# Autodesk Inventor assembly: Extruder 2.3
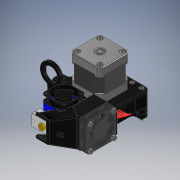
[picture p0: Inventor's stored thumbnail of the model, 180x180]
Saved by Autodesk Inventor 2020.2 (Build 242310000, 310)
## iProperties
Created: 2020-03-20
Part Number: Extruder 2.3
Document SubType Name: Assembly
Designer: rah75
Author: rah75
## Documents named in this file (29)
- C:\Users\rah75\Documents\GitHub\LETU-Maker\CAD\Autodesk Inventor\Modules_6001-9999\Extruder\Assemblies\Extruder_LM6012.iam
- C:\Users\rah75\Documents\GitHub\LETU-Maker\CAD\Autodesk Inventor\Modules_6001-9999\Extruder\Printed_Parts\Extruder_Lower_Block_LM6008.ipt
- C:\Users\rah75\Documents\GitHub\LETU-Maker\CAD\Autodesk Inventor\Modules_6001-9999\Extruder\Printed_Parts\Extruder_Motor_Plate_LM6009.ipt
- C:\Users\rah75\Documents\GitHub\LETU-Maker\CAD\Autodesk Inventor\Modules_6001-9999\Extruder\Printed_Parts\Extruder_Upper_Block_LM6011.ipt
- C:\Users\rah75\Documents\GitHub\LETU-Maker\CAD\Autodesk Inventor\Modules_6001-9999\Extruder\Printed_Parts\Extruder_Mount_Plate_LM6010.ipt
- C:\Users\rah75\Documents\GitHub\LETU-Maker\CAD\Autodesk Inventor\Stock_Components_1001-2999\Misc\Hot_End_Plate_LM1038.ipt
- C:\Users\rah75\Documents\GitHub\LETU-Maker\CAD\Autodesk Inventor\Stock_Components_1001-2999\Motors\NEMA_17_LM1028.ipt
- C:\Users\rah75\Documents\GitHub\LETU-Maker\CAD\Autodesk Inventor\Modules_6001-9999\Extruder\Printed_Parts\Extruder_Gear_0.8m57t_Internal_LM6004.ipt
- C:\Users\rah75\Documents\GitHub\LETU-Maker\CAD\Autodesk Inventor\Stock_Components_1001-2999\Power_Transmission\Bearings\625-ZZ_5x16mm_LM1030.ipt
- C:\Users\rah75\Documents\GitHub\LETU-Maker\CAD\Autodesk Inventor\Stock_Components_1001-2999\Power_Transmission\extruder_knob_11mm_LM1033.ipt
- C:\Users\rah75\Documents\GitHub\LETU-Maker\CAD\Autodesk Inventor\Modules_6001-9999\Extruder\Fabricated_Parts\Extruder_Fillament_Guide_LM6002.ipt
- C:\Users\rah75\Documents\GitHub\LETU-Maker\CAD\Autodesk Inventor\Stock_Components_1001-2999\Electrical\e3d-v6-hotend-3\e3d v6.iam
- C:\Users\rah75\Documents\GitHub\LETU-Maker\CAD\Autodesk Inventor\Modules_6001-9999\Extruder\Printed_Parts\Extruder_Pinion_0.8m12t_LM6005.ipt
- C:\Users\rah75\Documents\GitHub\LETU-Maker\CAD\Autodesk Inventor\Modules_6001-9999\Extruder\Fabricated_Parts\Extruder_Drive_Shaft_LM6001.ipt
- C:\Users\rah75\Documents\GitHub\LETU-Maker\CAD\Autodesk Inventor\Modules_6001-9999\Extruder\Fabricated_Parts\Extruder_Idler_Shaft_LM6003.ipt
- C:\Users\rah75\Documents\GitHub\LETU-Maker\CAD\Autodesk Inventor\Stock_Components_1001-2999\Fasteners\Screws\SHCS_m3x20_LM1014.ipt
- C:\Users\rah75\Documents\GitHub\LETU-Maker\CAD\Autodesk Inventor\Stock_Components_1001-2999\Fasteners\Screws\SHCS_m3x35_LM1011.ipt
- C:\Users\rah75\Documents\GitHub\LETU-Maker\CAD\Autodesk Inventor\Modules_6001-9999\Extruder\Printed_Parts\Extruder_Inductive_Sensor_Mount_LM6007.ipt
- C:\Users\rah75\Documents\GitHub\LETU-Maker\CAD\Autodesk Inventor\Stock_Components_1001-2999\Electrical\fan_40x40mm_LM1027.ipt
- C:\Users\rah75\Documents\GitHub\LETU-Maker\CAD\Autodesk Inventor\Stock_Components_1001-2999\Fasteners\Nuts\heat_insert_m3_LM1017.ipt
- C:\Users\rah75\Documents\GitHub\LETU-Maker\CAD\Autodesk Inventor\Stock_Components_1001-2999\Fasteners\Screws\SHCS_m3x8_LM1008.ipt
- C:\Users\rah75\Documents\GitHub\LETU-Maker\CAD\Autodesk Inventor\Stock_Components_1001-2999\Fasteners\Screws\SHCS_m3x10_LM1015.ipt
- C:\Users\rah75\Documents\GitHub\LETU-Maker\CAD\Autodesk Inventor\Stock_Components_1001-2999\Fasteners\Screws\SHCS_m3x30_LM1012.ipt
- C:\Users\rah75\Documents\GitHub\LETU-Maker\CAD\Autodesk Inventor\Stock_Components_1001-2999\Fasteners\Screws\SHCS_m3x12_LM1037.ipt
- C:\Users\rah75\Documents\GitHub\LETU-Maker\CAD\Autodesk Inventor\Stock_Components_1001-2999\Fasteners\Nuts\hex_nut_m3_LM1019.ipt
- C:\Users\rah75\Documents\GitHub\LETU-Maker\CAD\Autodesk Inventor\Stock_Components_1001-2999\Fasteners\Screws\Set Screws\set_screw_m3x6_LM1016.ipt
- C:\Users\rah75\Documents\GitHub\LETU-Maker\CAD\Autodesk Inventor\Stock_Components_1001-2999\Fasteners\Screws\SHCS_m3x5_LM1007.ipt
- C:\Users\rah75\Documents\GitHub\LETU-Maker\CAD\Autodesk Inventor\Modules_6001-9999\Extruder\Printed_Parts\Extruder_Fan_Duct_LM6006.ipt
- C:\Users\rah75\Documents\GitHub\LETU-Maker\CAD\Autodesk Inventor\Modules_6001-9999\Extruder\Printed_Parts\Extruder_Hot_End_Spacer_LM6014.ipt
## Components (50 placed, 28 different names)
1. Extruder_Lower_Block_LM6008:2 — Mate:4, Insert:3, Insert:5, Mate:9, Mate:10, Angle:1, Insert:11, Mate:21, Insert:20, Insert:25, Insert:44
2. Extruder_Motor_Plate_LM6009:2 — Mate:4, Insert:3, Insert:4, Mate:5, Mate:6, Insert:6, Mate:11, Insert:16, Insert:17, Insert:18, Insert:19, Insert:23, Insert:24, Insert:28, Insert:29, Insert:41, Insert:42
3. Extruder_Upper_Block_LM6011:1 — Insert:4, Mate:5, Insert:7, Mate:13, Mate:15, Angle:2, Mate:19, Insert:14, Insert:15, Insert:21, Insert:22, Insert:39, Insert:40
4. Extruder_Mount_Plate_LM6010:1 — Insert:5, Mate:6, Insert:8, Insert:30, Insert:31
5. Hot_End_Plate_LM1038:1 — Mate:9, Mate:10, Angle:1, Mate:20
6. NEMA_17_LM1028:1 — Insert:6, Mate:11, Mate:18, Flush:1, Angle:4, Angle:5
7. Extruder_Gear_0.8m57t_Internal_LM6004:1 — Insert:9, Insert:10, Insert:37, Mate:28, Insert:43
8. extruder_knob_11mm_LM1033:1 — Insert:10, Mate:12, Mate:16
9. Extruder_Fillament_Guide_LM6002:1 — Mate:15, Mate:16, Mate:17, Angle:2
10. e3d v6:1 [sub-assembly] — Insert:11, Angle:5
11. Extruder_Pinion_0.8m12t_LM6005:1 — Mate:18, Flush:1
12. Extruder_Drive_Shaft_LM6001:1 — Insert:12
13. Extruder_Idler_Shaft_LM6003:1 — Insert:13
14. Extruder_Inductive_Sensor_Mount_LM6007:2 — Mate:20, Mate:21, Angle:4, Insert:26
15. fan_40x40mm_LM1027:1 — Insert:33, Insert:34, Insert:35, Insert:36
16. Extruder_Fan_Duct_LM6006:1
17. Extruder_Hot_End_Spacer_LM6014:1 — Insert:44
18. 625-ZZ_5x16mm_LM1030:2 — Insert:8, Insert:9
19. 625-ZZ_5x16mm_LM1030:3 — Mate:12, Mate:13, Mate:17, Mate:19, Insert:13
20. 625-ZZ_5x16mm_LM1030:1 — Insert:7, Insert:12
21. hex_nut_m3_LM1019:3 — Insert:40
22. hex_nut_m3_LM1019:4 — Insert:39
23. SHCS_m3x5_LM1007:1 — Insert:42
24. SHCS_m3x5_LM1007:2 — Insert:41
25. heat_insert_m3_LM1017:1 — Insert:20, Mate:27
26. heat_insert_m3_LM1017:2 — Insert:22
27. heat_insert_m3_LM1017:3 — Insert:21
28. SHCS_m3x8_LM1008:1 — Insert:23
29. SHCS_m3x8_LM1008:2 — Insert:24
30. heat_insert_m3_LM1017:4 — Insert:25
31. SHCS_m3x10_LM1015:1 — Insert:26
32. SHCS_m3x10_LM1015:2 — Mate:27
33. heat_insert_m3_LM1017:5 — Insert:28
34. heat_insert_m3_LM1017:6 — Insert:29
35. SHCS_m3x30_LM1012:1 — Insert:30
36. SHCS_m3x30_LM1012:2 — Insert:31
37. SHCS_m3x12_LM1037:1 — Insert:33
38. SHCS_m3x12_LM1037:2 — Insert:34
39. SHCS_m3x12_LM1037:3 — Insert:35
40. SHCS_m3x12_LM1037:4 — Insert:36
41. hex_nut_m3_LM1019:1 — Insert:37, Flush:6
42. hex_nut_m3_LM1019:2 — Insert:43, Mate:29, Flush:5
43. set_screw_m3x6_LM1016:1 — Mate:28, Flush:6
44. set_screw_m3x6_LM1016:2 — Mate:29, Flush:5
45. SHCS_m3x20_LM1014:2 — Insert:14
46. SHCS_m3x35_LM1011:1 — Insert:18
47. SHCS_m3x35_LM1011:2 — Insert:17
48. SHCS_m3x35_LM1011:3 — Insert:16
49. SHCS_m3x35_LM1011:4 — Insert:19
50. SHCS_m3x20_LM1014:1 — Insert:15
## Relationships (69: Insert 41, Mate 20, Angle 4, Flush 4)
- Mate:4: Extruder_Lower_Block_LM6008:2 ↔ Extruder_Motor_Plate_LM6009:2
- Insert:3: Extruder_Lower_Block_LM6008:2 ↔ Extruder_Motor_Plate_LM6009:2
- Insert:4: Extruder_Motor_Plate_LM6009:2 ↔ Extruder_Upper_Block_LM6011:1
- Mate:5: Extruder_Motor_Plate_LM6009:2 ↔ Extruder_Upper_Block_LM6011:1
- Insert:5: Extruder_Lower_Block_LM6008:2 ↔ Extruder_Mount_Plate_LM6010:1
- Mate:6: Extruder_Motor_Plate_LM6009:2 ↔ Extruder_Mount_Plate_LM6010:1
- Mate:9: Extruder_Lower_Block_LM6008:2 ↔ Hot_End_Plate_LM1038:1
- Mate:10: Extruder_Lower_Block_LM6008:2 ↔ Hot_End_Plate_LM1038:1
- Angle:1 (0 deg): Extruder_Lower_Block_LM6008:2 ↔ Hot_End_Plate_LM1038:1
- Insert:6: Extruder_Motor_Plate_LM6009:2 ↔ NEMA_17_LM1028:1
- Mate:11: Extruder_Motor_Plate_LM6009:2 ↔ NEMA_17_LM1028:1
- Insert:7: Extruder_Upper_Block_LM6011:1 ↔ 625-ZZ_5x16mm_LM1030:1
- Insert:8: Extruder_Mount_Plate_LM6010:1 ↔ 625-ZZ_5x16mm_LM1030:2
- Insert:9 (0.5 mm): Extruder_Gear_0.8m57t_Internal_LM6004:1 ↔ 625-ZZ_5x16mm_LM1030:2
- Insert:10 (1.5 mm): Extruder_Gear_0.8m57t_Internal_LM6004:1 ↔ extruder_knob_11mm_LM1033:1
- Mate:12: extruder_knob_11mm_LM1033:1 ↔ 625-ZZ_5x16mm_LM1030:3
- Mate:13 (0.25 mm): Extruder_Upper_Block_LM6011:1 ↔ 625-ZZ_5x16mm_LM1030:3
- Mate:15: Extruder_Upper_Block_LM6011:1 ↔ Extruder_Fillament_Guide_LM6002:1
- Mate:16: extruder_knob_11mm_LM1033:1 ↔ Extruder_Fillament_Guide_LM6002:1
- Mate:17: Extruder_Fillament_Guide_LM6002:1 ↔ 625-ZZ_5x16mm_LM1030:3
- Angle:2 (0 deg): Extruder_Upper_Block_LM6011:1 ↔ Extruder_Fillament_Guide_LM6002:1
- Insert:11: Extruder_Lower_Block_LM6008:2 ↔ e3d v6:1
- Mate:18: NEMA_17_LM1028:1 ↔ Extruder_Pinion_0.8m12t_LM6005:1
- Flush:1 (-0.75 mm): NEMA_17_LM1028:1 ↔ Extruder_Pinion_0.8m12t_LM6005:1
- Insert:12: Extruder_Drive_Shaft_LM6001:1 ↔ 625-ZZ_5x16mm_LM1030:1
- Mate:19: Extruder_Upper_Block_LM6011:1 ↔ 625-ZZ_5x16mm_LM1030:3
- Insert:13 (-4.5 mm): Extruder_Idler_Shaft_LM6003:1 ↔ 625-ZZ_5x16mm_LM1030:3
- Insert:14 (3 mm): Extruder_Upper_Block_LM6011:1 ↔ SHCS_m3x20_LM1014:2
- Insert:15 (3 mm): Extruder_Upper_Block_LM6011:1 ↔ SHCS_m3x20_LM1014:1
- Insert:16: Extruder_Motor_Plate_LM6009:2 ↔ SHCS_m3x35_LM1011:3
- Insert:17: Extruder_Motor_Plate_LM6009:2 ↔ SHCS_m3x35_LM1011:2
- Insert:18: Extruder_Motor_Plate_LM6009:2 ↔ SHCS_m3x35_LM1011:1
- Insert:19: Extruder_Motor_Plate_LM6009:2 ↔ SHCS_m3x35_LM1011:4
- Mate:20: Hot_End_Plate_LM1038:1 ↔ Extruder_Inductive_Sensor_Mount_LM6007:2
- Mate:21: Extruder_Lower_Block_LM6008:2 ↔ Extruder_Inductive_Sensor_Mount_LM6007:2
- Angle:4 (180 deg): NEMA_17_LM1028:1 ↔ Extruder_Inductive_Sensor_Mount_LM6007:2
- Angle:5 (0 deg): NEMA_17_LM1028:1 ↔ e3d v6:1
- [Flush]: Extruder_Lower_Block_LM6008:2 ↔ Extruder_Fan_Duct_LM6006:1
- [Mate]: Hot_End_Plate_LM1038:1 ↔ Extruder_Fan_Duct_LM6006:1
- Insert:20: Extruder_Lower_Block_LM6008:2 ↔ heat_insert_m3_LM1017:1
- Insert:21: Extruder_Upper_Block_LM6011:1 ↔ heat_insert_m3_LM1017:3
- Insert:22: Extruder_Upper_Block_LM6011:1 ↔ heat_insert_m3_LM1017:2
- Insert:23: Extruder_Motor_Plate_LM6009:2 ↔ SHCS_m3x8_LM1008:1
- Insert:24: Extruder_Motor_Plate_LM6009:2 ↔ SHCS_m3x8_LM1008:2
- Insert:25: Extruder_Lower_Block_LM6008:2 ↔ heat_insert_m3_LM1017:4
- Insert:26 (-4 mm): Extruder_Inductive_Sensor_Mount_LM6007:2 ↔ SHCS_m3x10_LM1015:1
- [Insert]: Extruder_Fan_Duct_LM6006:1 ↔ SHCS_m3x10_LM1015:2
- Insert:28: Extruder_Motor_Plate_LM6009:2 ↔ heat_insert_m3_LM1017:5
- Insert:29: Extruder_Motor_Plate_LM6009:2 ↔ heat_insert_m3_LM1017:6
- Insert:30: Extruder_Mount_Plate_LM6010:1 ↔ SHCS_m3x30_LM1012:1
- Insert:31: Extruder_Mount_Plate_LM6010:1 ↔ SHCS_m3x30_LM1012:2
- [Insert]: fan_40x40mm_LM1027:1 ↔ Extruder_Fan_Duct_LM6006:1
- [Mate]: fan_40x40mm_LM1027:1 ↔ Extruder_Fan_Duct_LM6006:1
- Mate:27: heat_insert_m3_LM1017:1 ↔ SHCS_m3x10_LM1015:2
- Insert:33: fan_40x40mm_LM1027:1 ↔ SHCS_m3x12_LM1037:1
- Insert:34: fan_40x40mm_LM1027:1 ↔ SHCS_m3x12_LM1037:2
- Insert:35: fan_40x40mm_LM1027:1 ↔ SHCS_m3x12_LM1037:3
- Insert:36: fan_40x40mm_LM1027:1 ↔ SHCS_m3x12_LM1037:4
- Insert:37: Extruder_Gear_0.8m57t_Internal_LM6004:1 ↔ hex_nut_m3_LM1019:1
- Mate:28: Extruder_Gear_0.8m57t_Internal_LM6004:1 ↔ set_screw_m3x6_LM1016:1
- Insert:39: Extruder_Upper_Block_LM6011:1 ↔ hex_nut_m3_LM1019:4
- Insert:40: Extruder_Upper_Block_LM6011:1 ↔ hex_nut_m3_LM1019:3
- Insert:41: Extruder_Motor_Plate_LM6009:2 ↔ SHCS_m3x5_LM1007:2
- Insert:42: Extruder_Motor_Plate_LM6009:2 ↔ SHCS_m3x5_LM1007:1
- Insert:43: Extruder_Gear_0.8m57t_Internal_LM6004:1 ↔ hex_nut_m3_LM1019:2
- Mate:29: hex_nut_m3_LM1019:2 ↔ set_screw_m3x6_LM1016:2
- Flush:5 (2.5 mm): hex_nut_m3_LM1019:2 ↔ set_screw_m3x6_LM1016:2
- Flush:6 (2.5 mm): hex_nut_m3_LM1019:1 ↔ set_screw_m3x6_LM1016:1
- Insert:44: Extruder_Lower_Block_LM6008:2 ↔ Extruder_Hot_End_Spacer_LM6014:1
